# Autodesk Inventor assembly: ADSK-MH-10012
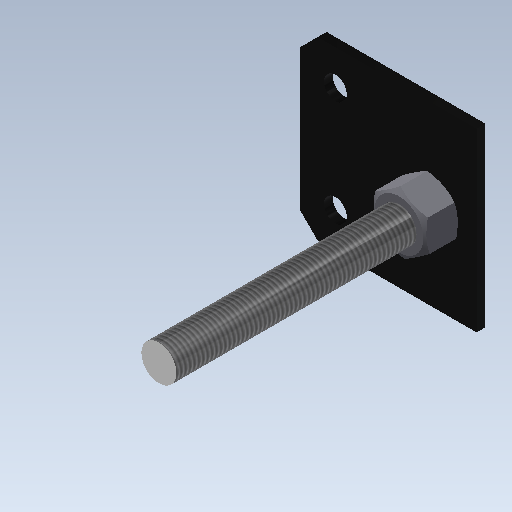
[picture p0: Inventor's stored thumbnail of the model, 512x512]
Saved by Autodesk Inventor 2021.1 (Build 251245010, 245A)
## iProperties
Created: 2008-03-10
Part Number: ADSK-MH-10012
Document SubType Name: Assembly
Designer: R.O'mahony
Description: Foot Assembly
Engineer: Demir Ali
Checked By: Demir Ali
Company: Autodesk Ltd
Author: R.O'mahony
Keywords: Roller Conveyor
Revision Number: A
## Documents named in this file (4)
- C:\Users\peter\source\repos\InventorDA-FLC\Dataset\Discharge Conveyor\ADSK-MH-10012.iam
- C:\Users\peter\source\repos\InventorDA-FLC\Dataset\Discharge Conveyor\ADSK-MH-10042.ipt
- C:\Users\peter\source\repos\InventorDA-FLC\Dataset\Discharge Conveyor\ISO 4034 - M20ISO.ipt
- C:\Users\peter\source\repos\InventorDA-FLC\Dataset\Discharge Conveyor\ADSK-MH-10041.ipt
## Components (3 placed, 3 different names)
1. ADSK-MH-10042:1 — Insert:1, Flush:1, Insert:2
2. ISO 4034 M20:1 — Insert:1
3. ADSK-MH-10041:1 — Flush:1, Insert:2
## Relationships (3: Insert 2, Flush 1)
- Flush:1: ADSK-MH-10042:1 ↔ ADSK-MH-10041:1
- Insert:1: ADSK-MH-10042:1 ↔ ISO 4034 M20:1
- Insert:2: ADSK-MH-10042:1 ↔ ADSK-MH-10041:1
